# Autodesk Inventor assembly: FemaleHeaderPin_2x3_90
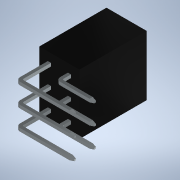
[picture p0: Inventor's stored thumbnail of the model, 180x180]
Saved by Autodesk Inventor 2021 (Build 250183000, 183)
## iProperties
Created: 2021-09-29
Part Number: FemaleHeaderPin_2x3_90
Document SubType Name: Assembly
Designer: ermoz
Author: ermoz
## Documents named in this file (2)
- D:\Moje Wyczyny\My_Poor_Projects\Sneak100_MiniSumo\minisumo-sneak100\mechanics\ElectricElements\FemaleHeaderPin_2x3_90.iam
- D:\Moje Wyczyny\My_Poor_Projects\Sneak100_MiniSumo\minisumo-sneak100\mechanics\ElectricElements\FemaleHederPin_2_90.ipt
## Components (3 placed, 1 different names)
1. FemaleHederPin_2_90:1 — Flush:1, Flush:4, Mate:2
2. FemaleHederPin_2_90:2 — Flush:1, Flush:2, Flush:3, Flush:4, Mate:1, Mate:2
3. FemaleHederPin_2_90:3 — Flush:2, Flush:3, Mate:1
## Relationships (6: Flush 4, Mate 2)
- Flush:1: FemaleHederPin_2_90:1 ↔ FemaleHederPin_2_90:2
- Flush:2: FemaleHederPin_2_90:2 ↔ FemaleHederPin_2_90:3
- Flush:3: FemaleHederPin_2_90:2 ↔ FemaleHederPin_2_90:3
- Flush:4: FemaleHederPin_2_90:1 ↔ FemaleHederPin_2_90:2
- Mate:1: FemaleHederPin_2_90:2 ↔ FemaleHederPin_2_90:3
- Mate:2: FemaleHederPin_2_90:1 ↔ FemaleHederPin_2_90:2
